# Autodesk Inventor assembly: 42146-00
(part 2 of 3)
408. 6558-Blue:55 — Einfügen:345, Passend:154
409. 6558-Blue:56 — Einfügen:346
410. 6558-Blue:57 — Einfügen:348
411. 6558-Blue:58 — Einfügen:349
412. 6558-Blue:59 — Einfügen:347
413. 2780-Black:100 — Einfügen:351
414. 32525-Yellow:3 — Einfügen:351, Einfügen:353, Einfügen:393, Passend:242
415. 32525-Yellow:4 — Einfügen:352, Einfügen:394, Passend:241
416. 6558-Blue:62 — Einfügen:374, Passend:237
417. 6558-Blue:63 — Einfügen:373, Passend:236
418. 32073-LtBluishGray:3 — Einfügen:375, Passend:235, Passend:238
419. 60484-Yellow:3 — Einfügen:373, Einfügen:374, Einfügen:376, Einfügen:377, Einfügen:378
420. 79768-DkBluishGray:1 — Einfügen:378, Passend:236, Einfügen:380, Einfügen:435, Winkel:10
421. 6536-Yellow:1 — Einfügen:375, Einfügen:376, Einfügen:381
422. 6536-Yellow:2 — Einfügen:377, Passend:235
423. 60484-Yellow:4 — Einfügen:380, Passend:237
424. 6536-Yellow:3 — Passend:238, Passend:239
425. 77765-MediumStoneGrey:7 — Einfügen:383
426. 77765-MediumStoneGrey:8 — Einfügen:382
427. 77765-MediumStoneGrey:9 — Einfügen:384
428. 32525-LtBluishGray:1 — Einfügen:385, Passend:240
429. 32054-LtBluishGray:25 — Einfügen:387
430. 32054-LtBluishGray:26 — Einfügen:386
431. 32054-LtBluishGray:23 — Einfügen:355
432. 2780-Black:101 — Einfügen:357, Passend:158
433. 2780-Black:102 — Einfügen:358
434. 2780-Black:103 — Einfügen:359
435. 2780-Black:104 — Einfügen:361, Passend:159
436. 6558-Blue:60 — Einfügen:360
437. 67491-Yellow:13 — Einfügen:371, Passend:161, Einfügen:552, Passend:454
438. 32524-Yellow:4 — Einfügen:355, Einfügen:366, Passend:157
439. 32524-Yellow:5 — Einfügen:361, Einfügen:362
440. 771710-Black:3 — Einfügen:357, Einfügen:358, Einfügen:359, Einfügen:370, Passend:159, Passend:160, Einfügen:551, Winkel:17
441. 32054-LtBluishGray:24 — Einfügen:356
442. 32524-Yellow:6 — Einfügen:356, Einfügen:367, Passend:156
443. 18654-Black:2 — Einfügen:360, Einfügen:362, Einfügen:368
444. 2780-Black:105 — Passend:160
445. 6558-Blue:61
446. 32524-Yellow:7
447. 18654-Black:3 — Einfügen:369
448. 85824 - HUB:1 [sub-assembly] — Einfügen:372, Passend:162
449. 2780-Black:106 — Einfügen:389, Passend:242
450. 2780-Black:107 — Einfügen:392
451. 2780-Black:108 — Einfügen:391, Passend:241
452. 2780-Black:109 — Einfügen:390
453. 44294-Yellow:1 — Einfügen:396
454. 44294-Yellow:2 — Einfügen:397
455. 2637-LtBluishGray:1 — Einfügen:401, Fluchtend:4, Einfügen:406, Fluchtend:9
456. 2637-LtBluishGray:2 — Fluchtend:5, Einfügen:402, Einfügen:410
457. 6632-LtBluishGray:1 — Einfügen:398, Einfügen:399, Fluchtend:4, Fluchtend:5, Fluchtend:6, Fluchtend:7
458. 6632-LtBluishGray:2 — Einfügen:400, Passend:246, Einfügen:401, Einfügen:402
459. 32449-Yellow:1 — Einfügen:407, Einfügen:408, Einfügen:410
460. 32449-Yellow:2 — Einfügen:409, Passend:248, Fluchtend:7, Einfügen:411, Fluchtend:8
461. 32062-Red:1 — Einfügen:398, Einfügen:400
462. 32062-Red:2 — Einfügen:399, Passend:246
463. 4519-Yellow:1 — Einfügen:407, Passend:248
464. 6632-LtBluishGray:3 — Einfügen:406, Fluchtend:6, Passend:249
465. 6632-LtBluishGray:4
466. 32062-Red:3
467. 32062-Red:4
468. 32062-Red:5 — Einfügen:408, Einfügen:409
469. 2637-LtBluishGray:3 — Einfügen:412, Fluchtend:9, Passend:249
470. 2637-LtBluishGray:4 — Einfügen:415, Passend:419, Winkel:4, Winkel:5, Einfügen:420, Passend:418, Passend:420, Passend:421
471. 2637-LtBluishGray:5 — Einfügen:416, Einfügen:419, Passend:419
472. 3707-Black:1 — Einfügen:413
473. 32184-Yellow:1 — Einfügen:413, Einfügen:414, Einfügen:415, Einfügen:416, Winkel:4, Einfügen:422
474. 48989-LtBluishGray:1 — Passend:418, Winkel:5, Einfügen:431, Passend:256, Winkel:8, Passend:420, Passend:421
475. 3707-Black:2 — Einfügen:414, Passend:251, Passend:252, Passend:254, Passend:255
476. 32184-Yellow:2 — Einfügen:419, Passend:252, Einfügen:423, Einfügen:425, Winkel:6
477. 32184-Yellow:3 — Einfügen:420, Passend:251, Einfügen:421, Einfügen:424, Einfügen:426
478. 18654-DkBluishGray:2 — Einfügen:421
479. 18654-DkBluishGray:3 — Einfügen:422
480. 3713-LtBluishGray:5 — Einfügen:424, Einfügen:428
481. 3713-LtBluishGray:6 — Einfügen:423, Einfügen:427
482. 32278-LtBluishGray:3 — Einfügen:426, Passend:253, Passend:423
483. 32278-LtBluishGray:2 — Einfügen:425, Winkel:6, Passend:253
484. 6632-LtBluishGray:5 — Einfügen:427, Passend:255
485. 6632-LtBluishGray:6 — Einfügen:428, Passend:254
486. 2637-LtBluishGray:6 — Einfügen:431
487. 2637-LtBluishGray:7 — Passend:256
488. 48989-LtBluishGray:2 — Winkel:8, Einfügen:432, Winkel:9, Einfügen:433
489. 32524-LtBluishGray:1 — Einfügen:432, Winkel:9, Einfügen:434, Winkel:10, Einfügen:436, Passend:422
490. 32524-LtBluishGray:2 — Einfügen:433, Passend:422
491. 6558-Blue:64 — Einfügen:434, Einfügen:436, Einfügen:435
492. 6558-Blue:69
493. 6558-Blue:70 — Passend:427
494. 40490-Yellow:3 — Einfügen:450
495. 6558-Blue:71
496. 6558-Blue:72 — Passend:428
497. 40490-Yellow:4 — Einfügen:451
498. 18939-LIGHTGREY:1 — Einfügen:443, Einfügen:442, Einfügen:441, Einfügen:445, Einfügen:450, Einfügen:451
499. 18939-LIGHTGREY:2 — Einfügen:444, Passend:425, Passend:424, Passend:427, Passend:428
500. 40490-Yellow:1 — Einfügen:437, Einfügen:438, Einfügen:442
501. 40490-Yellow:2 — Einfügen:441
502. 6558-Blue:65 — Einfügen:437, Passend:424
503. 6558-Blue:66 — Einfügen:438
504. 6558-Blue:67 — Passend:425
505. 6558-Blue:68 — Passend:426
506. 44294-Yellow:3 — Einfügen:485
507. 44294-Yellow:4 — Einfügen:486
508. 2637-LtBluishGray:8
509. 2637-LtBluishGray:9
510. 41677-LtBluishGray:1
511. 41677-LtBluishGray:2
512. 4519-Yellow:2
513. 4519-Yellow:3
514. 6538c-Red:1
515. 4519-Yellow:4
516. 4519-Yellow:5
517. 6538c-Red:2
518. 32449-Yellow:3
519. 11478-LtBluishGray:1 — Fluchtend:14
520. 43093-Blue:19
521. 43093-Blue:20
522. 32073-LtBluishGray:4 — Passend:435
523. 32073-LtBluishGray:5
524. 42610-LtBluishGray:1
525. 42610-LtBluishGray:2
526. 42610-LtBluishGray:3
527. 26287-LtBluishGray:1
528. 2637-LtBluishGray:10
529. 2637-LtBluishGray:11
530. 41677-LtBluishGray:3
531. 32449-Yellow:4
532. 11478-LtBluishGray:2
533. 41677-LtBluishGray:4
534. 32062-Red:6
535. 32062-Red:7
536. 92907-LtBluishGray:1
537. 32062-Red:8
538. 32062-Red:9
539. 92907-LtBluishGray:2
540. 32073-LtBluishGray:8
541. 11478-LtBluishGray:4
542. 32449-Yellow:6
543. 26287-LtBluishGray:2
544. 42610-LtBluishGray:6
545. 42610-LtBluishGray:5
546. 42610-LtBluishGray:4
547. 32073-LtBluishGray:7
548. 32073-LtBluishGray:6
549. 43093-Blue:22
550. 43093-Blue:21
551. 11478-LtBluishGray:3
552. 32449-Yellow:5
553. 32062-Red:11
554. 6536-Yellow:4
555. 6632-LtBluishGray:8 — Winkel:23
556. 6632-LtBluishGray:7
557. 32062-Red:12
558. 42610-LtBluishGray:10
559. 6536-Yellow:5
560. 77765-MediumStoneGrey:10
561. 77765-MediumStoneGrey:11
562. 3706-Red:2 — Passend:449
563. 41677-LtBluishGray:6 — Einfügen:538
564. 3713-LtBluishGray:7 — Einfügen:540, Einfügen:541
565. 62462-Yellow:1 — Einfügen:539
566. 62462-Yellow:2 — Einfügen:539, Einfügen:540
567. 32449-Yellow:7
568. 11478-LtBluishGray:5
569. 43093-Blue:23
570. 43093-Blue:24
571. 32073-LtBluishGray:9
572. 42610-LtBluishGray:7
573. 42610-LtBluishGray:8
574. 42610-LtBluishGray:9
575. 26287-LtBluishGray:3
576. 32449-Yellow:8
577. 11478-LtBluishGray:6
578. 3706-Red:1 — Einfügen:538
579. 41677-LtBluishGray:5 — Passend:449, Einfügen:541
580. 32073-LtBluishGray:10
581. 64179-Red:2
582. 4274-Red:1
583. 64179-Red:1
584. 58176-TransRed:1
585. 4274-Red:2
586. 58176-TransRed:2
587. 6558-Blue:73
588. 6558-Blue:74
589. 11214-Red:13
590. 11214-Red:14
591. 64179-Red:3
592. 32054-LtBluishGray:27
593. 32054-LtBluishGray:28
594. 32054-LtBluishGray:29
595. 32054-LtBluishGray:30
596. 32054-LtBluishGray:31 — Einfügen:548, Einfügen:549, Einfügen:551
597. 4519-LtBluishGray:1 — Einfügen:548
598. 32062-Red:10 — Einfügen:545
599. 41677-DKBluishGray:1 — Einfügen:545, Einfügen:546, Passend:453, Einfügen:549
600. 41677-DKBluishGray:2 — Einfügen:546, Passend:453, Einfügen:547, Winkel:15, Einfügen:550, Winkel:16, Winkel:17
601. 25214-LtBluishGray:1 — Einfügen:547, Winkel:15
602. 25214-LtBluishGray:2 — Einfügen:550, Winkel:16
603. 4274-Red:3
604. 4274-Red:4
605. 4274-Red:5
606. 4274-Red:6
607. 32524-Yellow:8 — Einfügen:557, Passend:455, Passend:468, Passend:469, Passend:470
608. 4162-LtBluishGray:1 — Passend:468, Passend:469, Passend:470, Passend:472, Fluchtend:31
609. 4162-LtBluishGray:2
610. 4162-LtBluishGray:3
611. 3022-Yellow:1 — Passend:473
612. 3710-Yellow:1 — Passend:474
613. 2420-Yellow:1 — Fluchtend:32
614. 4162-LtBluishGray:4 — Passend:472, Fluchtend:31
615. 4162-LtBluishGray:5
616. 3022-Yellow:2
617. 3022-Yellow:3
618. 3020-Yellow:1
619. 3020-Yellow:2 — Passend:471
620. 44873-LtBluishGray:1 — Einfügen:559, Einfügen:560
621. 44873-LtBluishGray:2 — Einfügen:558, Einfügen:561
622. 87994-LtBluishGray:1 — Einfügen:561, Passend:478
623. 87994-LtBluishGray:2 — Einfügen:560, Passend:477
624. 63037-LtBluishGray:1 — Einfügen:558, Passend:476
625. 63037-LtBluishGray:2 — Einfügen:559, Passend:475
626. 44873-LtBluishGray:3 — Einfügen:562, Passend:478
627. 63965-LtBluishGray:1 — Einfügen:562, Einfügen:563
628. 43093-Blue:25 — Einfügen:568, Einfügen:575
629. 4274-LtBluishGray:1 — Einfügen:564, Passend:481
630. 4274-LtBluishGray:2 — Einfügen:565, Passend:480
631. 3023-Black:1 — Passend:479, Passend:480, Passend:481, Passend:482, Passend:483, Fluchtend:34, Fluchtend:35, Fluchtend:42
632. 54200-TransClear:1 — Passend:482, Passend:484, Fluchtend:33, Fluchtend:35
633. 54200-TransClear:2 — Passend:483, Passend:484, Fluchtend:33, Fluchtend:34
634. 32291-DkBluishGray:1 — Einfügen:564, Einfügen:565, Passend:479, Einfügen:572
635. 4274-LtBluishGray:3
636. 4274-LtBluishGray:4
637. 3023-Black:2 — Fluchtend:42
638. 54200-TransClear:3
639. 54200-TransClear:4
640. 32291-DkBluishGray:2 — Einfügen:568, Passend:497
641. 43093-Blue:26 — Einfügen:573
642. 4274-LtBluishGray:5
643. 4274-LtBluishGray:6
644. 3023-Black:3 — Winkel:18
645. 54200-TransClear:5
646. 54200-TransClear:6
647. 32291-DkBluishGray:3
648. 43093-Blue:27 — Einfügen:572, Einfügen:574
## Relationships (989: Insert 581, Mate 341, Flush 42, Angle 23, RelateRotation 2)
- Winkel:19 [Angle] (-30 deg): 42146-03:1 ↔ 32278-Yellow:5
- Passend:249 [Mate] (-8 mm): 6632-LtBluishGray:3 ↔ 2637-LtBluishGray:3
- Einfügen:395 [Insert]: 42146-26:1 ↔ 42146-27:1
- Passend:418 [Mate] (8 mm): 2637-LtBluishGray:4 ↔ 48989-LtBluishGray:1
- Einfügen:436 [Insert]: 32524-LtBluishGray:1 ↔ 6558-Blue:64
- Einfügen:434 [Insert]: 32524-LtBluishGray:1 ↔ 6558-Blue:64
- Einfügen:452 [Insert]: 42146-28:1 ↔ 42146-29:1
- Passend:435 [Mate] (160 mm): 42146-27:1 ↔ 32073-LtBluishGray:4
- Einfügen:490 [Insert]: 42146-28:1 ↔ 42146-32:1
- Passend:440 [Mate] (-0.8 mm): 42146-28:1 ↔ 42146-32:1
- Passend:448 [Mate]: 42146-28:1 ↔ 42146-32:1
- Winkel:14 [Angle] (-40 deg): 42146-30:1 ↔ 42146-31:1
- Passend:1 [Mate]: 42146-01:1
- Passend:2 [Mate]: 42146-01:1
- Passend:3 [Mate]: 42146-01:1
- Fluchtend:1 [Flush] (-4 mm): 42146-01:1
- Einfügen:1 [Insert]: 42146-01:1 ↔ 42146-02:1
- Passend:4 [Mate]: 42146-01:1 ↔ 42146-02:1
- Einfügen:2 [Insert]: 42146-01:1 ↔ 42146-03:1
- Passend:5 [Mate]: 42146-01:1 ↔ 42146-03:1
- Einfügen:3 [Insert]: 42146-03:1 ↔ 32054-LtBluishGray:1
- Einfügen:4 [Insert]: 42146-02:1 ↔ 32054-LtBluishGray:2
- Einfügen:5 [Insert]: 42146-01:1 ↔ 43093-Blue:1
- Einfügen:6 [Insert]: 42146-01:1 ↔ 43093-Blue:2
- Einfügen:7 [Insert]: 42146-02:1 ↔ 42146-04:1
- Passend:6 [Mate]: 42146-03:1 ↔ 42146-04:1
- Einfügen:8 [Insert]: 42146-02:1 ↔ 42146-05:1
- Passend:7 [Mate]: 42146-03:1 ↔ 42146-05:1
- Einfügen:9 [Insert]: 6558-Blue:3 ↔ 32524-Yellow:1
- Einfügen:10 [Insert]: 6558-Blue:2 ↔ 32524-Yellow:1
- Einfügen:11 [Insert]: 6558-Blue:3 ↔ 73507-Black:2
- Einfügen:12 [Insert]: 73507-Black:1 ↔ 32524-Yellow:1
- Passend:8 [Mate]: 6558-Blue:2 ↔ 73507-Black:1
- Passend:9 [Mate]: 6558-Blue:2 ↔ 73507-Black:2
- Passend:10 [Mate]: 42146-01:1 ↔ 73507-Black:2
- Passend:11 [Mate]: 42146-01:1 ↔ 73507-Black:2
- Passend:12 [Mate]: 42146-01:1 ↔ 73507-Black:2
- Einfügen:13 [Insert]: 6558-Blue:4 ↔ 73507-Black:2
- Einfügen:14 [Insert]: 6558-Blue:1 ↔ 73507-Black:1
- Einfügen:15 [Insert]: 42146-01:1 ↔ 11214-Red:4
- Einfügen:16 [Insert]: 42146-01:1 ↔ 11214-Red:3
- Einfügen:17 [Insert]: 42146-01:1 ↔ 11214-Red:2
- Einfügen:18 [Insert]: 42146-01:1 ↔ 11214-Red:1
- Passend:13 [Mate]: 42146-01:1 ↔ 42146-06:1
- Passend:14 [Mate] (4 mm): 42146-05:1 ↔ 42146-06:1
- Einfügen:19 [Insert] (8 mm): 42146-05:1 ↔ 42146-07:1
- Einfügen:20 [Insert]: 42146-01:1 ↔ 32054-LtBluishGray:7
- Einfügen:21 [Insert]: 42146-01:1 ↔ 32054-LtBluishGray:8
- Einfügen:22 [Insert]: 42146-01:1 ↔ 32054-LtBluishGray:9
- Einfügen:23 [Insert]: 42146-01:1 ↔ 32054-LtBluishGray:10
- Einfügen:24 [Insert]: 42146-01:1 ↔ 32054-LtBluishGray:6
- Einfügen:25 [Insert]: 42146-01:1 ↔ 32054-LtBluishGray:3
- Einfügen:26 [Insert]: 42146-01:1 ↔ 32054-LtBluishGray:4
- Einfügen:27 [Insert]: 42146-01:1 ↔ 32054-LtBluishGray:5
- Einfügen:28 [Insert]: 42146-01:1 ↔ 42146-08:1 - beweglich
- Passend:15 [Mate]: 42146-08:1 - beweglich ↔ 32054-LtBluishGray:8
- Einfügen:29 [Insert]: 32525-Red:1 ↔ 2780-Black:1
- Einfügen:30 [Insert]: 32525-Red:1 ↔ 2780-Black:2
- Passend:32 [Mate]: 42146-07:1 ↔ 32278-Yellow:5
- Passend:34 [Mate]: 42146-07:1 ↔ 32278-Yellow:4
- Einfügen:33 [Insert]: 42146-07:1 ↔ 32278-Yellow:3
- Passend:36 [Mate]: 42146-07:1 ↔ 32278-Yellow:2
- Einfügen:35 [Insert]: 32278-Yellow:4 ↔ 2780-Black:1
- Passend:16 [Mate]: 32278-Yellow:4 ↔ 2780-Black:2
- Passend:17 [Mate]: 42146-07:1 ↔ 32278-Yellow:2
- Passend:18 [Mate]: 42146-07:1 ↔ 32278-Yellow:5
- Passend:19 [Mate]: 42146-07:1 ↔ 32278-Yellow:4
- Passend:20 [Mate] (-3.6 mm): 42146-07:1 ↔ 32278-Yellow:3
- Einfügen:36 [Insert] (7.2 mm): 24316-ReddishBrown:1 ↔ 46372-LtBluishGray:1
- Einfügen:37 [Insert] (7.2 mm): 24316-ReddishBrown:2 ↔ 46372-LtBluishGray:2
- Einfügen:38 [Insert]: 32278-Yellow:1 ↔ 24316-ReddishBrown:2
- Einfügen:39 [Insert]: 32278-Yellow:1 ↔ 24316-ReddishBrown:1
- Einfügen:40 [Insert]: 6558-Blue:4 ↔ 32278-Yellow:1
- Passend:21 [Mate]: 6558-Blue:1 ↔ 32278-Yellow:1
- Drehung:1 [RelateRotation] (0.2 ul): 42146-07:1 ↔ 46372-LtBluishGray:2
- Drehung:2 [RelateRotation] (0.2 ul): 42146-07:1 ↔ 46372-LtBluishGray:1
- Einfügen:41 [Insert]: 15458-DkBluishGray:1 ↔ 6558-Blue:6
- Einfügen:42 [Insert]: 15458-DkBluishGray:1 ↔ 6558-Blue:5
- [Insert]: 15458-DkBluishGray:3 ↔ 6558-Blue:8
- [Insert]: 15458-DkBluishGray:3 ↔ 6558-Blue:7
- Einfügen:45 [Insert]: 42146-08:1 - beweglich ↔ 15458-DkBluishGray:3
- Passend:22 [Mate]: 42146-08:1 - beweglich ↔ 6558-Blue:8
- Einfügen:46 [Insert]: 42146-08:1 - beweglich ↔ 15458-DkBluishGray:1
- Passend:23 [Mate]: 42146-08:1 - beweglich ↔ 6558-Blue:6
- Einfügen:47 [Insert]: 42146-08:1 - beweglich ↔ 15458-DkBluishGray:2
- Passend:24 [Mate]: 15458-DkBluishGray:2 ↔ 6558-Blue:6
- Einfügen:48 [Insert]: 15458-DkBluishGray:3 ↔ 2780-Black:4
- Einfügen:49 [Insert]: 15458-DkBluishGray:3 ↔ 2780-Black:5
- Einfügen:50 [Insert]: 15458-DkBluishGray:2 ↔ 2780-Black:6
- Einfügen:51 [Insert]: 15458-DkBluishGray:2 ↔ 2780-Black:8
- Einfügen:52 [Insert]: 15458-DkBluishGray:1 ↔ 2780-Black:3
- Einfügen:53 [Insert]: 15458-DkBluishGray:1 ↔ 2780-Black:7
- Einfügen:54 [Insert]: 15458-DkBluishGray:3 ↔ 2780-Black:11
- Einfügen:55 [Insert]: 15458-DkBluishGray:2 ↔ 2780-Black:10
- Einfügen:56 [Insert]: 15458-DkBluishGray:1 ↔ 2780-Black:9
- Einfügen:57 [Insert]: 32278-Yellow:4 ↔ 67491-Yellow:1
- Passend:25 [Mate]: 42146-07:1 ↔ 67491-Yellow:1
- Passend:33 [Mate]: 42146-07:1 ↔ 32278-Yellow:5
- Passend:35 [Mate]: 42146-07:1 ↔ 32278-Yellow:4
- Passend:37 [Mate]: 42146-07:1 ↔ 32278-Yellow:2
- Einfügen:58 [Insert]: 32278-Yellow:4 ↔ 67491-Yellow:2
- Passend:38 [Mate]: 42146-07:1 ↔ 67491-Yellow:2
- Einfügen:59 [Insert]: 15458-DkBluishGray:1 ↔ 40490-LtBluishGray:1
- Passend:39 [Mate]: 2780-Black:5 ↔ 40490-LtBluishGray:1
- Einfügen:60 [Insert]: 32525-Red:1 ↔ 39790-Black:1
- Passend:40 [Mate]: 32525-Red:1 ↔ 39790-Black:1
- Einfügen:61 [Insert]: 32054-LtBluishGray:11 ↔ 39790-Black:1
- Einfügen:62 [Insert]: 32054-LtBluishGray:12 ↔ 39790-Black:1
- Einfügen:63 [Insert]: 67491-Yellow:3 ↔ 6558-Blue:9
- Einfügen:64 [Insert]: 67491-Yellow:3 ↔ 6558-Blue:12
- Einfügen:65 [Insert]: 67491-Yellow:3 ↔ 6558-Blue:10
- Einfügen:66 [Insert]: 67491-Yellow:3 ↔ 6558-Blue:11
- [Insert]: 67491-Yellow:4 ↔ 6558-Blue:13
- [Insert]: 67491-Yellow:4 ↔ 6558-Blue:16
- [Insert]: 67491-Yellow:4 ↔ 6558-Blue:14
- [Insert]: 67491-Yellow:4 ↔ 6558-Blue:15
- Einfügen:71 [Insert]: 42146-02:1 ↔ 67491-Yellow:4
- Einfügen:72 [Insert]: 42146-03:1 ↔ 67491-Yellow:3
- Passend:41 [Mate]: 42146-03:1 ↔ 67491-Yellow:3
- Passend:42 [Mate]: 42146-02:1 ↔ 67491-Yellow:4
- Einfügen:73 [Insert]: 67491-Yellow:4 ↔ 6558-Blue:17
- Einfügen:74 [Insert]: 42146-02:1 ↔ 18651-Black:1
- Einfügen:75 [Insert]: 67491-Yellow:4 ↔ 18654-DkBluishGray:1
- Einfügen:76 [Insert]: 42146-09:1 ↔ 67491-Yellow:4
- Passend:43 [Mate]: 42146-09:1 ↔ 67491-Yellow:4
- Einfügen:77 [Insert]: 32140-LtBluishGray:1 ↔ 6558-Blue:19
- Einfügen:78 [Insert]: 32140-LtBluishGray:1 ↔ 6558-Blue:18
- Einfügen:79 [Insert]: 32140-LtBluishGray:1 ↔ 2780-Black:12
- Einfügen:80 [Insert]: 42146-09:1 ↔ 32140-LtBluishGray:1
- Passend:44 [Mate]: 42146-09:1 ↔ 6558-Blue:18
- Einfügen:81 [Insert]: 42146-10:1 ↔ 67491-Yellow:3
- Passend:45 [Mate]: 42146-10:1 ↔ 6558-Blue:9
- Einfügen:82 [Insert]: 32140-LtBluishGray:2 ↔ 6558-Blue:21
- Einfügen:83 [Insert]: 32140-LtBluishGray:2 ↔ 6558-Blue:20
- Einfügen:84 [Insert]: 32140-LtBluishGray:2 ↔ 2780-Black:13
- Einfügen:85 [Insert]: 42146-10:1 ↔ 32140-LtBluishGray:2
- Passend:46 [Mate]: 42146-10:1 ↔ 6558-Blue:20
- Einfügen:86 [Insert]: 42146-09:1 ↔ 32278-LtBluishGray:1
- Passend:47 [Mate]: 42146-10:1 ↔ 32278-LtBluishGray:1
- Einfügen:87 [Insert]: 42146-09:1 ↔ 32054-LtBluishGray:14
- Einfügen:88 [Insert]: 42146-10:1 ↔ 32054-LtBluishGray:13
- Einfügen:89 [Insert]: 18654-DkBluishGray:1 ↔ 43857-LtBluishGray:1
- Passend:48 [Mate]: 18651-Black:1 ↔ 43857-LtBluishGray:1
- Einfügen:90 [Insert]: 32278-Yellow:6 ↔ 2780-Black:14
- Einfügen:91 [Insert]: 32278-Yellow:6 ↔ 2780-Black:15
- Einfügen:92 [Insert]: 42146-10:1 ↔ 32278-Yellow:6
- Passend:49 [Mate]: 42146-09:1 ↔ 2780-Black:15
- Einfügen:93 [Insert]: 42146-10:1 ↔ 11214-Red:5
- Einfügen:94 [Insert]: 42146-09:1 ↔ 11214-Red:6
- Einfügen:95 [Insert]: 42146-10:1 ↔ 32054-LtBluishGray:15
- Einfügen:96 [Insert]: 42146-09:1 ↔ 32054-LtBluishGray:16
- Einfügen:97 [Insert]: 42146-10:1 ↔ 6558-Blue:23
- Einfügen:98 [Insert]: 42146-09:1 ↔ 6558-Blue:22
- Einfügen:99 [Insert]: 42146-10:1 ↔ 6558-Blue:24
- Einfügen:100 [Insert]: 42146-09:1 ↔ 6558-Blue:25
- Einfügen:101 [Insert]: 42146-09:1 ↔ 42146-11:1
- Passend:50 [Mate]: 42146-11:1 ↔ 6558-Blue:23
- Einfügen:102 [Insert]: 42146-11:1 ↔ 32054-LtBluishGray:19
- Einfügen:103 [Insert]: 42146-11:1 ↔ 32054-LtBluishGray:18
- Einfügen:104 [Insert]: 42146-11:1 ↔ 32054-LtBluishGray:17
- Einfügen:105 [Insert]: 42146-11:1 ↔ 32054-LtBluishGray:20
- Passend:51 [Mate]: 2780-Black:9 ↔ 39790-Black:1
- Einfügen:106 [Insert]: 42146-09:1 ↔ 42146-12:1
- Passend:52 [Mate]: 42146-09:1 ↔ 42146-12:1
- Einfügen:107 [Insert]: 2780-Black:17 ↔ 32524-Yellow:2
- Einfügen:108 [Insert]: 2780-Black:16 ↔ 6629-DkBluishGray:1
- Einfügen:109 [Insert]: 43093-Blue:4 ↔ 6629-DkBluishGray:1
- Einfügen:110 [Insert]: 43093-Blue:3 ↔ 6629-DkBluishGray:1
- Passend:53 [Mate]: 43093-Blue:3 ↔ 6629-DkBluishGray:1
- Einfügen:111 [Insert]: 42146-12:1 ↔ 6629-DkBluishGray:1
- Passend:54 [Mate]: 42146-12:1 ↔ 2780-Black:16
- Einfügen:112 [Insert]: 42146-12:1 ↔ 32524-Yellow:2
- Passend:55 [Mate]: 42146-12:1 ↔ 32524-Yellow:2
- Einfügen:113 [Insert]: 42146-10:1 ↔ 42146-13:1
- Passend:56 [Mate]: 42146-10:1 ↔ 42146-13:1
- [Insert]: 2780-Black:19 ↔ 32524-Yellow:3
- Einfügen:115 [Insert]: 2780-Black:18 ↔ 6629-DkBluishGray:2
- Einfügen:116 [Insert]: 43093-Blue:6 ↔ 6629-DkBluishGray:2
- Einfügen:117 [Insert]: 43093-Blue:5 ↔ 6629-DkBluishGray:2
- [Mate]: 43093-Blue:5 ↔ 6629-DkBluishGray:2
- Einfügen:118 [Insert]: 42146-13:1 ↔ 32524-Yellow:3
- Passend:58 [Mate]: 42146-13:1 ↔ 32524-Yellow:3
- Einfügen:119 [Insert]: 42146-13:1 ↔ 6629-DkBluishGray:2
- Einfügen:120 [Insert]: 42146-13:1 ↔ 43093-Blue:6
- Einfügen:121 [Insert]: 42146-09:1 ↔ 42146-14:1
- Passend:59 [Mate]: 42146-09:1 ↔ 42146-14:1
- Einfügen:122 [Insert]: 6558-Blue:26 ↔ 32316-LtBluishGray:2
- Einfügen:123 [Insert]: 6558-Blue:27 ↔ 32316-LtBluishGray:2
- Einfügen:124 [Insert] (7.2 mm): 6589-Tan:1 ↔ 15462-ReddishBrown:1
- Einfügen:125 [Insert]: 6589-Tan:1 ↔ 62462-LtBluishGray:1
- Einfügen:126 [Insert]: 6589-Tan:2 ↔ 62462-LtBluishGray:1
- Einfügen:127 [Insert]: 2780-Black:20 ↔ 32316-LtBluishGray:2
- Einfügen:128 [Insert]: 32316-LtBluishGray:1 ↔ 32316-LtBluishGray:2
- Passend:60 [Mate]: 6558-Blue:27 ↔ 32316-LtBluishGray:1
- Einfügen:129 [Insert]: 15462-ReddishBrown:1 ↔ 32316-LtBluishGray:1
- Einfügen:130 [Insert]: 42146-09:1 ↔ 32316-LtBluishGray:2
- Passend:61 [Mate]: 42146-14:1 ↔ 6558-Blue:27
- Einfügen:131 [Insert]: 11214-Red:7 ↔ 60483-DkBluishGray:1
- Einfügen:132 [Insert]: 2780-Black:21 ↔ 60483-DkBluishGray:1
- Einfügen:133 [Insert]: 60483-DkBluishGray:1 ↔ 32316-DkBluishGray:1
- Einfügen:134 [Insert]: 2780-Black:22 ↔ 32316-DkBluishGray:1
- Einfügen:135 [Insert]: 18945-DkBluishGray:1 ↔ 32316-DkBluishGray:1
- Passend:62 [Mate]: 2780-Black:21 ↔ 32316-DkBluishGray:1
- Passend:63 [Mate]: 2780-Black:22 ↔ 18945-DkBluishGray:1
- Einfügen:136 [Insert]: 2780-Black:23 ↔ 18945-DkBluishGray:1
- Einfügen:137 [Insert]: 6558-Blue:28 ↔ 18945-DkBluishGray:1
- Einfügen:138 [Insert]: 18945-DkBluishGray:1 ↔ 771710-DkBluishGray:1
- Passend:64 [Mate]: 2780-Black:23 ↔ 771710-DkBluishGray:1
- Einfügen:139 [Insert] (7.2 mm): 24316-ReddishBrown:3 ↔ 3713-LtBluishGray:1
- Einfügen:140 [Insert]: 771710-DkBluishGray:1 ↔ 24316-ReddishBrown:3
- Einfügen:141 [Insert]: 771710-DkBluishGray:1 ↔ 2780-Black:25
- Einfügen:142 [Insert]: 771710-DkBluishGray:1 ↔ 32316-DkBluishGray:2
- Passend:65 [Mate]: 771710-DkBluishGray:1 ↔ 32316-DkBluishGray:2
- Einfügen:143 [Insert]: 6558-Blue:29 ↔ 11947-DkBluishGray:1
- Einfügen:144 [Insert]: 2780-Black:24 ↔ 11947-DkBluishGray:1
- Einfügen:145 [Insert]: 32316-DkBluishGray:2 ↔ 11947-DkBluishGray:1
- Passend:66 [Mate]: 2780-Black:24 ↔ 32316-DkBluishGray:2
- Einfügen:146 [Insert]: 42146-09:1 ↔ 771710-DkBluishGray:1
- Passend:67 [Mate]: 42146-09:1 ↔ 771710-DkBluishGray:1
- Passend:68 [Mate]: 42146-14:1 ↔ 24316-ReddishBrown:3
- [Insert]: 2780-Black:26 ↔ 6629-DkBluishGray:3
- [Insert]: 43093-Blue:8 ↔ 6629-DkBluishGray:3
- [Insert]: 43093-Blue:7 ↔ 6629-DkBluishGray:3
- [Mate]: 43093-Blue:7 ↔ 6629-DkBluishGray:3
- Einfügen:150 [Insert]: 18945-DkBluishGray:1 ↔ 6629-DkBluishGray:3
- Passend:70 [Mate]: 18945-DkBluishGray:1 ↔ 2780-Black:26
- Einfügen:151 [Insert]: 42146-10:1 ↔ 42146-15:1
- Passend:71 [Mate]: 42146-10:1 ↔ 42146-15:1
- [Insert]: 6558-Blue:30 ↔ 32316-LtBluishGray:4
- [Insert]: 6558-Blue:31 ↔ 32316-LtBluishGray:4
- [Insert] (7.2 mm): 6589-Tan:3 ↔ 15462-ReddishBrown:2
- [Insert]: 6589-Tan:3 ↔ 62462-LtBluishGray:2
- [Insert]: 6589-Tan:4 ↔ 62462-LtBluishGray:2
- [Insert]: 2780-Black:27 ↔ 32316-LtBluishGray:4
- [Insert]: 32316-LtBluishGray:3 ↔ 32316-LtBluishGray:4
- [Mate]: 6558-Blue:31 ↔ 32316-LtBluishGray:3
- [Insert]: 15462-ReddishBrown:2 ↔ 32316-LtBluishGray:3
- [Insert]: 11214-Red:8 ↔ 60483-DkBluishGray:2
- [Insert]: 2780-Black:28 ↔ 60483-DkBluishGray:2
- [Insert]: 60483-DkBluishGray:2 ↔ 32316-DkBluishGray:3
- [Insert]: 2780-Black:29 ↔ 32316-DkBluishGray:3
- [Insert]: 18945-DkBluishGray:2 ↔ 32316-DkBluishGray:3
- [Mate]: 2780-Black:28 ↔ 32316-DkBluishGray:3
- [Mate]: 2780-Black:29 ↔ 18945-DkBluishGray:2
- [Insert]: 2780-Black:30 ↔ 18945-DkBluishGray:2
- [Insert]: 6558-Blue:32 ↔ 18945-DkBluishGray:2
- [Insert]: 18945-DkBluishGray:2 ↔ 771710-DkBluishGray:2
- [Mate]: 2780-Black:30 ↔ 771710-DkBluishGray:2
- [Insert] (7.2 mm): 24316-ReddishBrown:4 ↔ 3713-LtBluishGray:2
- Einfügen:169 [Insert]: 771710-DkBluishGray:2 ↔ 24316-ReddishBrown:4
- [Insert]: 771710-DkBluishGray:2 ↔ 2780-Black:32
- [Insert]: 771710-DkBluishGray:2 ↔ 32316-DkBluishGray:4
- [Mate]: 771710-DkBluishGray:2 ↔ 32316-DkBluishGray:4
- Einfügen:172 [Insert]: 6558-Blue:33 ↔ 11946-DkBluishGray:1
- Einfügen:173 [Insert]: 2780-Black:31 ↔ 11946-DkBluishGray:1
- Einfügen:174 [Insert]: 32316-DkBluishGray:4 ↔ 11946-DkBluishGray:1
- [Mate]: 2780-Black:31 ↔ 32316-DkBluishGray:4
- Einfügen:175 [Insert]: 2780-Black:33 ↔ 6629-DkBluishGray:4
- Einfügen:176 [Insert]: 43093-Blue:10 ↔ 6629-DkBluishGray:4
- Einfügen:177 [Insert]: 43093-Blue:9 ↔ 6629-DkBluishGray:4
- [Mate]: 43093-Blue:9 ↔ 6629-DkBluishGray:4
- Einfügen:178 [Insert]: 18945-DkBluishGray:2 ↔ 6629-DkBluishGray:4
- Passend:79 [Mate]: 18945-DkBluishGray:2 ↔ 2780-Black:33
- Einfügen:179 [Insert]: 42146-15:1 ↔ 32316-LtBluishGray:3
- Passend:80 [Mate]: 42146-10:1 ↔ 6558-Blue:30
- Einfügen:180 [Insert]: 42146-10:1 ↔ 771710-DkBluishGray:2
- Passend:81 [Mate]: 42146-10:1 ↔ 771710-DkBluishGray:2
- Einfügen:181 [Insert]: 42146-09:1 ↔ 42146-16:2
- Passend:82 [Mate]: 42146-09:1 ↔ 42146-16:2
- Einfügen:182 [Insert]: 42146-10:1 ↔ 42146-16:1
- Passend:83 [Mate]: 42146-10:1 ↔ 42146-16:1
- Einfügen:183 [Insert]: 42146-09:1 ↔ 42146-17:1
- Passend:84 [Mate]: 42146-09:1 ↔ 42146-17:1
- Einfügen:184 [Insert]: 42146-10:1 ↔ 42146-17:2
- Passend:85 [Mate]: 42146-10:1 ↔ 42146-17:2
- [Insert]: 2780-Black:34 ↔ 6629-DkBluishGray:5
- [Insert]: 43093-Blue:12 ↔ 6629-DkBluishGray:5
- [Insert]: 43093-Blue:11 ↔ 6629-DkBluishGray:5
- [Mate]: 43093-Blue:11 ↔ 6629-DkBluishGray:5
- Einfügen:188 [Insert]: 42146-13:1 ↔ 6629-DkBluishGray:5
- Passend:87 [Mate]: 42146-13:1 ↔ 2780-Black:34
- [Insert]: 2780-Black:35 ↔ 6629-DkBluishGray:6
- [Insert]: 43093-Blue:14 ↔ 6629-DkBluishGray:6
- [Insert]: 43093-Blue:13 ↔ 6629-DkBluishGray:6
- [Mate]: 43093-Blue:13 ↔ 6629-DkBluishGray:6
- Einfügen:192 [Insert]: 42146-12:1 ↔ 6629-DkBluishGray:6
- Passend:89 [Mate]: 42146-12:1 ↔ 2780-Black:35
- Einfügen:193 [Insert]: 18945-DkBluishGray:1 ↔ 2780-Black:39
- Einfügen:194 [Insert]: 18945-DkBluishGray:1 ↔ 2780-Black:38
- Einfügen:195 [Insert]: 42146-09:1 ↔ 2780-Black:36
- Einfügen:196 [Insert]: 42146-09:1 ↔ 2780-Black:37
- Einfügen:197 [Insert]: 42146-09:1 ↔ 2780-Black:41
- Einfügen:198 [Insert]: 42146-09:1 ↔ 2780-Black:40
- Einfügen:199 [Insert]: 42146-10:1 ↔ 2780-Black:46
- Einfügen:200 [Insert]: 42146-10:1 ↔ 2780-Black:47
- Einfügen:201 [Insert]: 42146-10:1 ↔ 2780-Black:42
- Einfügen:202 [Insert]: 42146-10:1 ↔ 2780-Black:43
- Einfügen:203 [Insert]: 18945-DkBluishGray:2 ↔ 2780-Black:44
- Einfügen:204 [Insert]: 18945-DkBluishGray:2 ↔ 2780-Black:45
- Einfügen:205 [Insert]: 42146-10:1 ↔ 40490-DkBluishGray:1
- Einfügen:206 [Insert]: 42146-10:1 ↔ 40490-DkBluishGray:2
- Einfügen:207 [Insert]: 42146-09:1 ↔ 40490-DkBluishGray:4
- Einfügen:208 [Insert]: 42146-09:1 ↔ 40490-DkBluishGray:3
- Passend:90 [Mate]: 42146-13:1 ↔ 40490-DkBluishGray:2
- Passend:91 [Mate]: 2780-Black:45 ↔ 40490-DkBluishGray:1
- Passend:92 [Mate]: 2780-Black:39 ↔ 40490-DkBluishGray:4
- Passend:93 [Mate]: 42146-12:1 ↔ 40490-DkBluishGray:3
- Einfügen:209 [Insert]: 42146-15:1 ↔ 42146-18:1
- Passend:94 [Mate]: 42146-15:1 ↔ 42146-18:1
- Passend:95 [Mate] (12.4 mm): 42146-13:1 ↔ 42146-19:1
- Passend:96 [Mate]: 42146-19:1 ↔ 24316-ReddishBrown:4
- Winkel:1 [Angle] (0 deg): 42146-19:1 ↔ 771710-DkBluishGray:2
- Passend:97 [Mate]: 42146-19:2 ↔ 24316-ReddishBrown:3
- Winkel:2 [Angle] (0 deg): 42146-19:2 ↔ 771710-DkBluishGray:1
- Passend:98 [Mate] (12.4 mm): 42146-19:2 ↔ 18945-DkBluishGray:1
- Einfügen:210 [Insert]: 42146-20:1 ↔ 67491-Yellow:1
- Passend:99 [Mate]: 42146-20:1 ↔ 67491-Yellow:1
- Einfügen:211 [Insert]: 42146-20:1 ↔ 6558-Blue:34
- Einfügen:212 [Insert]: 42146-20:1 ↔ 6558-Blue:37
- Einfügen:213 [Insert]: 42146-20:1 ↔ 6558-Blue:38
- Einfügen:214 [Insert]: 42146-20:1 ↔ 6558-Blue:35
- Einfügen:215 [Insert]: 42146-20:1 ↔ 6558-Blue:36
- Einfügen:216 [Insert]: 42146-20:1 ↔ 11214-Red:10
- Einfügen:217 [Insert]: 42146-20:1 ↔ 11214-Red:9
- Einfügen:218 [Insert]: 42146-20:1 ↔ 2780-Black:48
- Einfügen:219 [Insert]: 42146-20:1 ↔ 2780-Black:49
- Einfügen:220 [Insert]: 42146-20:1 ↔ 2780-Black:51
- Einfügen:221 [Insert]: 42146-20:1 ↔ 2780-Black:50
- Einfügen:222 [Insert]: 67491-Yellow:5 ↔ 6558-Blue:39
- Einfügen:223 [Insert]: 67491-Yellow:5 ↔ 2780-Black:52
- Einfügen:224 [Insert]: 67491-Yellow:5 ↔ 2780-Black:54
- Einfügen:225 [Insert]: 67491-Yellow:5 ↔ 2780-Black:53
- Einfügen:226 [Insert]: 42146-20:1 ↔ 67491-Yellow:5
- Passend:100 [Mate]: 6558-Blue:35 ↔ 67491-Yellow:5
- Einfügen:227 [Insert]: 42146-20:1 ↔ 40490-LtBluishGray:2
- Passend:101 [Mate]: 2780-Black:48 ↔ 40490-LtBluishGray:2
- Einfügen:228 [Insert]: 42146-20:1 ↔ 6558-Blue:40
- Einfügen:229 [Insert]: 42146-20:1 ↔ 6558-Blue:43
- Einfügen:230 [Insert]: 42146-20:1 ↔ 2780-Black:56
- Einfügen:231 [Insert]: 42146-20:1 ↔ 11214-Red:11
- Einfügen:232 [Insert]: 42146-20:1 ↔ 11214-Red:12
- Einfügen:233 [Insert]: 42146-20:1 ↔ 6558-Blue:44
- Einfügen:234 [Insert]: 42146-20:1 ↔ 6558-Blue:41
- Einfügen:235 [Insert]: 42146-20:1 ↔ 6558-Blue:42
- Einfügen:236 [Insert]: 42146-20:1 ↔ 2780-Black:55
- Einfügen:237 [Insert]: 42146-20:1 ↔ 2780-Black:57
- Einfügen:238 [Insert]: 42146-20:1 ↔ 2780-Black:58
- Einfügen:239 [Insert]: 67491-Yellow:6 ↔ 6558-Blue:45
- Einfügen:240 [Insert]: 67491-Yellow:6 ↔ 2780-Black:59
- Einfügen:241 [Insert]: 67491-Yellow:6 ↔ 2780-Black:61
- Einfügen:242 [Insert]: 67491-Yellow:6 ↔ 2780-Black:60
- Einfügen:243 [Insert]: 42146-20:1 ↔ 40490-LtBluishGray:3
- Einfügen:244 [Insert]: 42146-20:1 ↔ 67491-Yellow:6
- Passend:102 [Mate]: 2780-Black:55 ↔ 40490-LtBluishGray:3
- Passend:103 [Mate]: 6558-Blue:41 ↔ 67491-Yellow:6
- Einfügen:245 [Insert]: 32526-Yellow:1 ↔ 2780-Black:62
- Einfügen:246 [Insert]: 32526-Yellow:2 ↔ 2780-Black:63
- Einfügen:247 [Insert]: 32526-Yellow:2 ↔ 6558-Blue:47
- Einfügen:248 [Insert]: 32526-Yellow:1 ↔ 6558-Blue:48
- Einfügen:249 [Insert]: 32526-Yellow:1 ↔ 6558-Blue:46
- Einfügen:250 [Insert]: 32526-Yellow:2 ↔ 6558-Blue:49
- Einfügen:251 [Insert]: 42146-20:1 ↔ 32526-Yellow:1
- Einfügen:252 [Insert]: 42146-20:1 ↔ 32526-Yellow:2
- Passend:104 [Mate]: 42146-20:1 ↔ 6558-Blue:49
- Passend:105 [Mate]: 42146-20:1 ↔ 6558-Blue:46
- Einfügen:253 [Insert]: 60484-Yellow:1 ↔ 3673-LtBluishGray:1
- Einfügen:254 [Insert]: 2780-Black:64 ↔ 60484-Yellow:1
- Einfügen:255 [Insert]: 2780-Black:65 ↔ 60484-Yellow:1
- [Insert]: 60484-Yellow:2 ↔ 3673-LtBluishGray:2
- [Insert]: 2780-Black:66 ↔ 60484-Yellow:2
- [Insert]: 2780-Black:67 ↔ 60484-Yellow:2
- Einfügen:259 [Insert]: 42146-20:1 ↔ 60484-Yellow:2
- Einfügen:260 [Insert]: 42146-20:1 ↔ 60484-Yellow:1
- Passend:106 [Mate]: 42146-20:1 ↔ 2780-Black:65
- Passend:107 [Mate]: 42146-20:1 ↔ 2780-Black:66
- [Insert]: 67491-Yellow:7 ↔ 2780-Black:68
- [Insert]: 67491-Yellow:7 ↔ 2780-Black:69
- Einfügen:263 [Insert]: 67491-Yellow:7 ↔ 2780-Black:70
- Einfügen:264 [Insert]: 67491-Yellow:7 ↔ 2780-Black:71
- [Insert]: 67491-Yellow:8 ↔ 2780-Black:74
- [Insert]: 67491-Yellow:8 ↔ 2780-Black:75
- [Insert]: 67491-Yellow:8 ↔ 2780-Black:76
- [Insert]: 67491-Yellow:8 ↔ 2780-Black:77
- Einfügen:269 [Insert]: 67491-Yellow:7 ↔ 2780-Black:73
- Einfügen:270 [Insert]: 67491-Yellow:7 ↔ 6558-Blue:50
- Einfügen:271 [Insert]: 67491-Yellow:7 ↔ 6558-Blue:51
- Einfügen:272 [Insert]: 67491-Yellow:7 ↔ 67491-Yellow:5
- Passend:108 [Mate]: 67491-Yellow:7 ↔ 6558-Blue:48
- Einfügen:273 [Insert]: 67491-Yellow:8 ↔ 67491-Yellow:9
- Passend:109 [Mate]: 2780-Black:74 ↔ 67491-Yellow:9
- Einfügen:274 [Insert]: 2780-Black:72 ↔ 67491-Yellow:8
- Einfügen:275 [Insert]: 67491-Yellow:9 ↔ 2780-Black:78
- Einfügen:276 [Insert]: 67491-Yellow:9 ↔ 6558-Blue:53
- Einfügen:277 [Insert]: 67491-Yellow:9 ↔ 6558-Blue:52
- Passend:110 [Mate]: 67491-Yellow:10 ↔ 6558-Blue:52
- Passend:111 [Mate]: 67491-Yellow:9 ↔ 67491-Yellow:10
- Passend:112 [Mate]: 67491-Yellow:10 ↔ 6558-Blue:53
- Einfügen:278 [Insert]: 67491-Yellow:9 ↔ 67491-Yellow:6
- Passend:113 [Mate]: 67491-Yellow:9 ↔ 2780-Black:59
- Einfügen:279 [Insert]: 42146-21:1 ↔ 67491-Yellow:8
- Passend:114 [Mate]: 42146-21:1 ↔ 67491-Yellow:8
- Einfügen:280 [Insert]: 771710-Black:1 ↔ 43093-Blue:15
- Einfügen:281 [Insert]: 771710-Black:1 ↔ 43093-Blue:16
- Einfügen:282 [Insert]: 771710-Black:1 ↔ 2780-Black:79
- Einfügen:283 [Insert]: 771710-Black:2 ↔ 43093-Blue:17
- Einfügen:284 [Insert]: 771710-Black:2 ↔ 43093-Blue:18
- [Insert]: 771710-Black:2 ↔ 2780-Black:80
- Einfügen:286 [Insert]: 771710-Black:1 ↔ 32002-Tan:2
- Einfügen:287 [Insert]: 32002-Tan:1 ↔ 771710-Black:2
- Einfügen:288 [Insert]: 60484-Yellow:1 ↔ 771710-Black:2
- Einfügen:289 [Insert]: 60484-Yellow:2 ↔ 771710-Black:1
- Einfügen:290 [Insert]: 771710-Black:1 ↔ 40490-LtBluishGray:4
- Einfügen:291 [Insert]: 771710-Black:2 ↔ 40490-LtBluishGray:4
- Einfügen:292 [Insert]: 2780-Black:81 ↔ 32278-Yellow:7
- Einfügen:293 [Insert]: 32054-LtBluishGray:21 ↔ 32278-Yellow:7
- [Insert]: 2780-Black:82 ↔ 32278-Yellow:8
- [Insert]: 32054-LtBluishGray:22 ↔ 32278-Yellow:8
- Einfügen:296 [Insert]: 42146-20:1 ↔ 32278-Yellow:7
- Einfügen:297 [Insert]: 42146-20:1 ↔ 32278-Yellow:8
- Passend:115 [Mate]: 42146-21:1 ↔ 32054-LtBluishGray:21
- Passend:116 [Mate]: 42146-21:1 ↔ 32054-LtBluishGray:22
- Einfügen:298 [Insert]: 67491-Yellow:7 ↔ 32525-Yellow:1
- Einfügen:299 [Insert]: 67491-Yellow:9 ↔ 32525-Yellow:2
- Passend:117 [Mate]: 42146-21:1 ↔ 32525-Yellow:2
- Passend:118 [Mate]: 42146-21:1 ↔ 32525-Yellow:1
- Passend:119 [Mate]: 18942-DkBluishGray:1 ↔ 18940-SandBlue:1
- Passend:120 [Mate]: 18942-DkBluishGray:1 ↔ 18940-SandBlue:1
- Einfügen:300 [Insert]: 32073-LtBluishGray:1 ↔ 32184-LtBluishGray:1
- Einfügen:301 [Insert] (-24 mm): 60485-LtBluishGray:1 ↔ 32184-LtBluishGray:1
- Passend:121 [Mate]: 18942-DkBluishGray:1 ↔ 77765-MediumStoneGrey:1
- Passend:122 [Mate]: 18942-DkBluishGray:1 ↔ 77765-MediumStoneGrey:2
- Passend:123 [Mate] (0.4 mm): 77765-MediumStoneGrey:1 ↔ 32184-LtBluishGray:2
- Passend:124 [Mate]: 18940-SandBlue:1 ↔ 77765-MediumStoneGrey:2
- Passend:125 [Mate]: 18654-Black:1 ↔ 77765-MediumStoneGrey:2
- Passend:126 [Mate]: 18940-SandBlue:1 ↔ 18654-Black:1
- Passend:127 [Mate] (-19.6 mm): 18940-SandBlue:1 ↔ 32073-LtBluishGray:1
- Passend:128 [Mate]: 18940-SandBlue:1 ↔ 77765-MediumStoneGrey:2
- Passend:129 [Mate]: 18942-DkBluishGray:1 ↔ 32073-LtBluishGray:1
- Passend:130 [Mate]: 18942-DkBluishGray:1 ↔ 60485-LtBluishGray:1
- Passend:131 [Mate] (4 mm): 18940-SandBlue:1 ↔ 32184-LtBluishGray:1
- Einfügen:302 [Insert]: 32184-LtBluishGray:1 ↔ 4265c-Yellow:1
- Fluchtend:2 [Flush]: 32184-LtBluishGray:1 ↔ 4265c-Yellow:1
- [Insert]: 32184-LtBluishGray:2 ↔ 4265c-Yellow:2
- [Flush]: 32184-LtBluishGray:2 ↔ 4265c-Yellow:2
- Passend:132 [Mate]: 60485-LtBluishGray:1 ↔ 32184-LtBluishGray:2
- Passend:133 [Mate]: 32073-LtBluishGray:1 ↔ 32184-LtBluishGray:2
- Passend:134 [Mate] (0.4 mm): 32184-LtBluishGray:1 ↔ 77765-MediumStoneGrey:1
- Einfügen:304 [Insert] (4 mm): 4265c-Yellow:1 ↔ 4265c-Yellow:4
- Einfügen:305 [Insert] (4 mm): 4265c-Yellow:2 ↔ 4265c-Yellow:3
- Einfügen:306 [Insert]: 32184-LtBluishGray:2 ↔ 6628-Red:1
- Einfügen:307 [Insert]: 32184-LtBluishGray:1 ↔ 6628-Red:2
- Einfügen:308 [Insert]: 4265c-Yellow:1 ↔ 32017-DKBluishGray:1
- Einfügen:309 [Insert]: 4265c-Yellow:2 ↔ 32017-DKBluishGray:2
- Einfügen:310 [Insert]: 3713-LtBluishGray:3 ↔ 60483-DkBluishGray:3
- Einfügen:311 [Insert]: 6558-Blue:54 ↔ 60483-DkBluishGray:3
- Einfügen:312 [Insert]: 32073-LtBluishGray:2 ↔ 3713-LtBluishGray:3
- [Insert]: 3713-LtBluishGray:4 ↔ 60483-DkBluishGray:4
- Einfügen:314 [Insert]: 32073-LtBluishGray:2 ↔ 3713-LtBluishGray:4
- Passend:135 [Mate]: 6558-Blue:54 ↔ 60483-DkBluishGray:4
- Einfügen:315 [Insert]: 18940-SandBlue:1 ↔ 60483-DkBluishGray:3
- Passend:136 [Mate]: 18940-SandBlue:1 ↔ 32073-LtBluishGray:2
- Einfügen:316 [Insert]: 42146-21:1 ↔ 18940-SandBlue:1
- Passend:137 [Mate]: 32017-DKBluishGray:1 ↔ 32002-Tan:1
- Passend:138 [Mate]: 32017-DKBluishGray:2 ↔ 32002-Tan:2
- Passend:139 [Mate] (-4 mm): 3713-LtBluishGray:3 ↔ 42146_70902_1:2
- Passend:140 [Mate] (-4 mm): 3713-LtBluishGray:4 ↔ 42146_70902_1:1
- Passend:141 [Mate]: 3713-LtBluishGray:4 ↔ 42146_70902_1:1
- Passend:142 [Mate]: 3713-LtBluishGray:3 ↔ 42146_70902_1:2
- Passend:143 [Mate]: 42146_70902_1:1 ↔ 42146_70902_1:2
- Winkel:3 [Angle] (-6.5 deg): 60483-DkBluishGray:4 ↔ 42146_70902_1:1
- Einfügen:317 [Insert]: 2780-Black:83 ↔ 67491-Yellow:11
- Einfügen:318 [Insert]: 67491-Yellow:7 ↔ 67491-Yellow:11
- Passend:144 [Mate]: 2780-Black:68 ↔ 67491-Yellow:11
- Passend:145 [Mate]: 42146-22:1 ↔ 67491-Yellow:8
- Passend:146 [Mate]: 42146-22:1 ↔ 67491-Yellow:8
- Passend:147 [Mate]: 42146-22:1 ↔ 67491-Yellow:11
- Einfügen:319 [Insert]: 67491-Yellow:8 ↔ 77765-MediumStoneGrey:6
- Einfügen:320 [Insert]: 67491-Yellow:8 ↔ 77765-MediumStoneGrey:5
- Einfügen:321 [Insert]: 67491-Yellow:11 ↔ 77765-MediumStoneGrey:4
- Einfügen:322 [Insert]: 67491-Yellow:11 ↔ 77765-MediumStoneGrey:3
- Einfügen:323 [Insert]: 42146-24:1 ↔ 67491-Yellow:8
- Einfügen:324 [Insert]: 42146-23:1 ↔ 67491-Yellow:11
- Passend:148 [Mate]: 42146-21:1 ↔ 42146-23:1
- Passend:149 [Mate]: 42146-21:1 ↔ 42146-24:1
- Einfügen:325 [Insert]: 43857-LtBluishGray:2 ↔ 2780-Black:85
- Einfügen:326 [Insert]: 43857-LtBluishGray:2 ↔ 2780-Black:84
- [Insert]: 43857-LtBluishGray:3 ↔ 2780-Black:87
- [Insert]: 43857-LtBluishGray:3 ↔ 2780-Black:86
- [Insert]: 43857-LtBluishGray:4 ↔ 2780-Black:89
- [Insert]: 43857-LtBluishGray:4 ↔ 2780-Black:88
- [Insert]: 43857-LtBluishGray:5 ↔ 2780-Black:91
- [Insert]: 43857-LtBluishGray:5 ↔ 2780-Black:90
- Einfügen:333 [Insert]: 67491-Yellow:11 ↔ 43857-LtBluishGray:5
- Einfügen:334 [Insert]: 67491-Yellow:11 ↔ 43857-LtBluishGray:4
- Einfügen:335 [Insert]: 67491-Yellow:8 ↔ 43857-LtBluishGray:2
- Einfügen:336 [Insert]: 67491-Yellow:8 ↔ 43857-LtBluishGray:3
- Passend:150 [Mate]: 42146-24:1 ↔ 2780-Black:87
- Passend:151 [Mate]: 42146-24:1 ↔ 2780-Black:85
- Passend:152 [Mate]: 42146-23:1 ↔ 2780-Black:91
- Passend:153 [Mate]: 42146-23:1 ↔ 2780-Black:89
- [Insert]: 2780-Black:92 ↔ 67491-Yellow:12
- Einfügen:338 [Insert]: 67491-Yellow:12 ↔ 2780-Black:93
- Einfügen:339 [Insert]: 67491-Yellow:12 ↔ 2780-Black:94
- Einfügen:340 [Insert]: 67491-Yellow:12 ↔ 2780-Black:95
- Einfügen:341 [Insert]: 67491-Yellow:12 ↔ 2780-Black:96